# Autodesk Inventor assembly: Diff
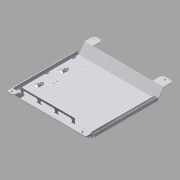
[picture p0: Inventor's stored thumbnail of the model, 180x180]
Saved by Autodesk Inventor 2017 (Build 210142000, 142)
## iProperties
Created: 2022-08-18
Part Number: Diff
Document SubType Name: Assembly
Designer: JTS
Author: JTS
## Documents named in this file (3)
- C:\Users\Windermac\Desktop\MASTER Honda Insight G1 IMA Bay\LiBCM003 - Battery Tray\Diff.iam
- C:\Users\Windermac\Desktop\MASTER Honda Insight G1 IMA Bay\LiBCM003 - Battery Tray\Prototype.ipt
- C:\Users\Windermac\Desktop\MASTER Honda Insight G1 IMA Bay\LiBCM003 - Battery Tray\47 Ah FoMoCo Aluminum Tray.ipt
## Components (2 placed, 2 different names)
1. Prototype:1 — Insert:1, Mate:1
2. 47 Ah FoMoCo Aluminum Tray:1 — Insert:1, Mate:1
## Relationships (2: Insert 1, Mate 1)
- Insert:1: Prototype:1 ↔ 47 Ah FoMoCo Aluminum Tray:1
- Mate:1: Prototype:1 ↔ 47 Ah FoMoCo Aluminum Tray:1
